# Autodesk Inventor assembly: Assembly_Cube_Flashlight_v3
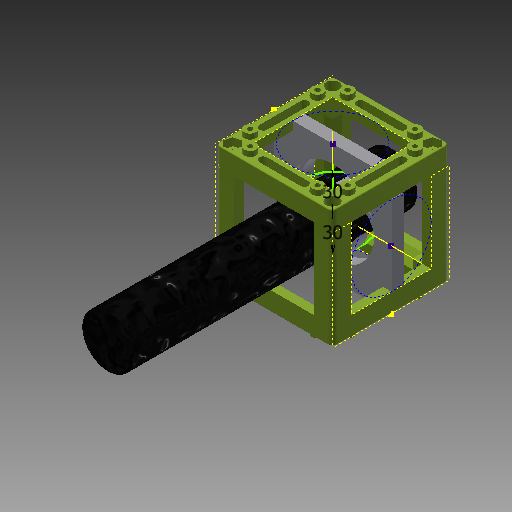
[picture p0: Inventor's stored thumbnail of the model, 512x512]
Saved by Autodesk Inventor 2019 (Build 230136000, 136)
## iProperties
Created: 2020-12-04
Part Number: Assembly_Cube_Flashlight_v3
Document SubType Name: Assembly
Designer: UC2
Author: UC2
## Documents named in this file (4)
- C:\Users\marsikovabarbora\Dropbox\UC2\02_CAD\INVENTOR\uc2_v3\Assembly_Cube_Flashlight_v3.iam
- C:\Users\marsikovabarbora\Dropbox\UC2\02_CAD\INVENTOR\uc2_v3\20_Cube_Insert_Holder-okular+flashlight_v3.ipt
- C:\Users\marsikovabarbora\Dropbox\UC2\02_CAD\INVENTOR\uc2_v3\Assembly_Cube_empty_IM_v3.iam
- C:\Users\marsikovabarbora\Dropbox\UC2\02_CAD\INVENTOR\uc2_v3\00_flashlight.ipt
## Components (3 placed, 3 different names)
1. 20_Cube_Insert_Holder-okular+flashlight_v3:1 — Fluchtend:1, Fluchtend:2, Passend:1
2. Assembly_Cube_empty_IM_v3:1 [sub-assembly] — Fluchtend:1, Fluchtend:2, Passend:1, Passend:2, Fluchtend:3
3. 00_flashlight:1 — Passend:2, Fluchtend:3
## Relationships (5: Flush 3, Mate 2)
- Fluchtend:1 [Flush]: 20_Cube_Insert_Holder-okular+flashlight_v3:1 ↔ Assembly_Cube_empty_IM_v3:1
- Fluchtend:2 [Flush]: 20_Cube_Insert_Holder-okular+flashlight_v3:1 ↔ Assembly_Cube_empty_IM_v3:1
- Passend:1 [Mate]: 20_Cube_Insert_Holder-okular+flashlight_v3:1 ↔ Assembly_Cube_empty_IM_v3:1
- Passend:2 [Mate]: Assembly_Cube_empty_IM_v3:1 ↔ 00_flashlight:1
- Fluchtend:3 [Flush]: Assembly_Cube_empty_IM_v3:1 ↔ 00_flashlight:1
